# Autodesk Inventor assembly: Body
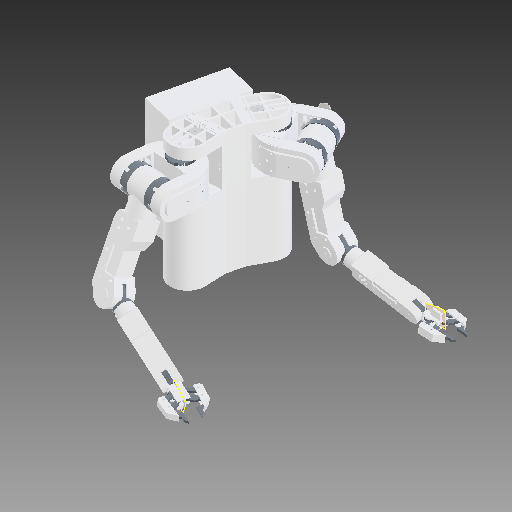
[picture p0: Inventor's stored thumbnail of the model, 512x512]
Saved by Autodesk Inventor 2017 SP1 (Build 210196100, 196)
## iProperties
Created: 2017-03-13
Part Number: Body
Document SubType Name: Assembly
Designer: zallen
Author: zallen
## Documents named in this file (3)
- C:\Users\Zach\Documents\GitHub\cr-laundry-robot\src\Body\Body.iam
- C:\Users\Zach\Documents\GitHub\cr-laundry-robot\src\Body\Arm Assembly\ArmAssembly.iam
- C:\Users\Zach\Documents\GitHub\cr-laundry-robot\src\Body\Chest Assembly\Chest Assembly.iam
## Components (3 placed, 2 different names)
1. ArmAssembly:1 [sub-assembly] — Mate:34, Mate:35, Mate:39
2. ArmAssembly:2 [sub-assembly] — Mate:19, Mate:32, Mate:40
3. Chest Assembly:1 [sub-assembly] — Mate:19, Mate:32, Mate:34, Mate:35, Mate:39, Mate:40, Mate:41
## Relationships (7: Mate 7)
- Mate:19: ArmAssembly:2 ↔ Chest Assembly:1
- Mate:32: ArmAssembly:2 ↔ Chest Assembly:1
- Mate:34: ArmAssembly:1 ↔ Chest Assembly:1
- Mate:35: ArmAssembly:1 ↔ Chest Assembly:1
- Mate:39: ArmAssembly:1 ↔ Chest Assembly:1
- Mate:40: ArmAssembly:2 ↔ Chest Assembly:1
- Mate:41: Chest Assembly:1
